# Autodesk Inventor assembly: ExplodedDiagram
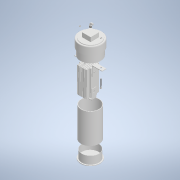
[picture p0: Inventor's stored thumbnail of the model, 180x180]
Saved by Autodesk Inventor 2020 (Build 240168000, 168)
## iProperties
Created: 2020-01-08
Part Number: ExplodedDiagram
Document SubType Name: Assembly
Designer: ellio
Author: ellio
## Documents named in this file (8)
- E:\TEMP BACKUP FOR MW\TEMPDOCS\hhogen\ExplodedDiagram.iam
- E:\TEMP BACKUP FOR MW\TEMPDOCS\hhogen\tubes\4in ID 7in length.ipt
- E:\TEMP BACKUP FOR MW\TEMPDOCS\hhogen\plumbing\Base Plug.ipt
- E:\TEMP BACKUP FOR MW\TEMPDOCS\hhogen\plumbing\4in Cleanout Adapter w Plug.ipt
- E:\TEMP BACKUP FOR MW\TEMPDOCS\hhogen\GeneratorPlateAssembly.iam
- E:\TEMP BACKUP FOR MW\TEMPDOCS\hhogen\2in Bolt w Nut.ipt
- E:\TEMP BACKUP FOR MW\TEMPDOCS\hhogen\Nut.ipt
- E:\TEMP BACKUP FOR MW\TEMPDOCS\hhogen\plumbing\Threaded Elbow.ipt
## Components (9 placed, 7 different names)
1. 4in ID 7in length:1 — Mate:1, Tangent:1, Mate:2, Tangent:2, Mate:4
2. Base Plug:1 — Mate:1, Tangent:1
3. 4in Cleanout Adapter w Plug:1 — Mate:2, Tangent:2, Mate:3, Mate:7, Mate:8
4. GeneratorPlateAssembly:1 [sub-assembly] — Mate:3, Mate:4, Mate:5, Tangent:3, Mate:6, Tangent:4, Insert:1, Insert:2
5. 2in Bolt w Nut:1 — Mate:5, Tangent:3
6. 2in Bolt w Nut:2 — Mate:6, Tangent:4
7. Nut:1 — Insert:2
8. Nut:2 — Insert:1
9. Threaded Elbow:1 — Mate:7, Mate:8
## Relationships (14: Mate 8, Tangent 4, Insert 2)
- Mate:1 (50.8 mm): 4in ID 7in length:1 ↔ Base Plug:1
- Tangent:1: 4in ID 7in length:1 ↔ Base Plug:1
- Mate:2 (254 mm): 4in ID 7in length:1 ↔ 4in Cleanout Adapter w Plug:1
- Tangent:2: 4in ID 7in length:1 ↔ 4in Cleanout Adapter w Plug:1
- Mate:3 (38.1 mm): 4in Cleanout Adapter w Plug:1 ↔ GeneratorPlateAssembly:1
- Mate:4 (-18.6944 mm): 4in ID 7in length:1 ↔ GeneratorPlateAssembly:1
- Mate:5 (50.8 mm): GeneratorPlateAssembly:1 ↔ 2in Bolt w Nut:1
- Tangent:3 (-2.286 mm): GeneratorPlateAssembly:1 ↔ 2in Bolt w Nut:1
- Mate:6 (50.8 mm): GeneratorPlateAssembly:1 ↔ 2in Bolt w Nut:2
- Tangent:4 (2.286 mm): GeneratorPlateAssembly:1 ↔ 2in Bolt w Nut:2
- Insert:1 (152.4 mm): GeneratorPlateAssembly:1 ↔ Nut:2
- Insert:2 (152.4 mm): GeneratorPlateAssembly:1 ↔ Nut:1
- Mate:7 (25.4 mm): 4in Cleanout Adapter w Plug:1 ↔ Threaded Elbow:1
- Mate:8: 4in Cleanout Adapter w Plug:1 ↔ Threaded Elbow:1
